# Autodesk Inventor assembly: 조립품1
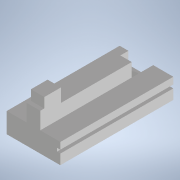
[picture p0: Inventor's stored thumbnail of the model, 180x180]
Saved by Autodesk Inventor 2020 (Build 240168000, 168)
## iProperties
Created: 2022-09-22
Part Number: 조립품1
Document SubType Name: Assembly
Designer: SeungJin
Author: SeungJin
## Documents named in this file (3)
- C:\Users\SeungJin\Documents\Inventor\CoMoVi\Package\조립품1.iam
- C:\Users\SeungJin\Documents\Inventor\CoMoVi\Package\center_tray_top.ipt
- C:\Users\SeungJin\Documents\Inventor\CoMoVi\Package\STO.ipt
## Components (2 placed, 2 different names)
1. center_tray_top:1 — 플러쉬:1, 플러쉬:2, 메이트:1
2. STO:1 — 플러쉬:1, 플러쉬:2, 메이트:1
## Relationships (3: Flush 2, Mate 1)
- 플러쉬:1 [Flush]: center_tray_top:1 ↔ STO:1
- 플러쉬:2 [Flush]: center_tray_top:1 ↔ STO:1
- 메이트:1 [Mate]: center_tray_top:1 ↔ STO:1
